# Autodesk Inventor assembly: Vex Traction Wheel 4x1
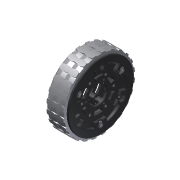
[picture p0: Inventor's stored thumbnail of the model, 180x180]
Saved by Autodesk Inventor 2013 (Build 170138000, 138)
## iProperties
Created: 2012-12-09
Part Number: Vex Traction Wheel 4x1
Document SubType Name: Assembly
Designer: Nemo
Mass: 137.424 g
Surface Area: 574.254 cm^2
Volume: 103.699 cm^3
Density: 1.32523 g/cm^3
Author: Nemo
## Documents named in this file (6)
- H:\Nemo\Documents\Robotics\COTS Parts\Wheels\VexPro Traction Wheels\Vex Traction Wheel 4x1.iam
- H:\Nemo\Documents\Robotics\COTS Parts\Wheels\VexPro Traction Wheels\Components\Traction Wheel Body 4in.ipt
- H:\Nemo\Documents\Robotics\COTS Parts\Fasteners\Hex Standoff 8-32 x750.ipt
- H:\Nemo\Documents\Robotics\COTS Parts\Fasteners\8-32 BHCS x1250.ipt
- H:\Nemo\Documents\Robotics\COTS Parts\Fasteners\8-32 locknut.ipt
- H:\Nemo\Documents\Robotics\COTS Parts\Wheels\VexPro Traction Wheels\Components\4 in Traction Tire.iam
## Components (16 placed, 5 different names)
1. Traction Wheel Body 4in:2 — Flush:1, Mate:2, Mate:4, Mate:5, Mate:6, Angle:1, Mate:7, Mate:8, Mate:9, Insert:4, Angle:3, Mate:11
2. Traction Wheel Body 4in:3 — Mate:5, Mate:8, Mate:9, Insert:3
3. 4 in Traction Tire:1 [sub-assembly] — Mate:10, Mate:11, Angle:4, Mate:13, Flush:2
4. 4 in Traction Tire:2 [sub-assembly] — Mate:12, Mate:13, Flush:2
5. Hex Standoff 8-32 x750:2 — Mate:6, Angle:1, Mate:7
6. Hex Standoff 8-32 x750:3
7. Hex Standoff 8-32 x750:4
8. Hex Standoff 8-32 x750:5
9. Hex Standoff 8-32 x750:6
10. Hex Standoff 8-32 x750:7
11. 8-32 BHCS x1250:1 — Insert:3
12. 8-32 locknut:2 — Insert:4, Angle:3
13. 8-32 BHCS x1250:3
14. 8-32 locknut:3
15. 8-32 BHCS x1250:5
16. 8-32 locknut:5
## Component patterns: (6 elements, first: Hex Standoff 8-32 x750:2), (3 elements, first: 8-32 BHCS x1250:1 + 8-32 locknut:2)
## Relationships (18: Mate 11, Angle 3, Flush 2, Insert 2)
- Flush:1: Traction Wheel Body 4in:2
- Mate:2: Traction Wheel Body 4in:2
- Mate:4: Traction Wheel Body 4in:2
- Mate:5: Traction Wheel Body 4in:2 ↔ Traction Wheel Body 4in:3
- Mate:6: Traction Wheel Body 4in:2 ↔ Hex Standoff 8-32 x750:2
- Angle:1 (0 deg): Traction Wheel Body 4in:2 ↔ Hex Standoff 8-32 x750:2
- Mate:7: Traction Wheel Body 4in:2 ↔ Hex Standoff 8-32 x750:2
- Mate:8: Traction Wheel Body 4in:2 ↔ Traction Wheel Body 4in:3
- Mate:9: Traction Wheel Body 4in:2 ↔ Traction Wheel Body 4in:3
- Insert:3: Traction Wheel Body 4in:3 ↔ 8-32 BHCS x1250:1
- Insert:4: Traction Wheel Body 4in:2 ↔ 8-32 locknut:2
- Angle:3 (0 deg): Traction Wheel Body 4in:2 ↔ 8-32 locknut:2
- Mate:10: 4 in Traction Tire:1
- Mate:11: Traction Wheel Body 4in:2 ↔ 4 in Traction Tire:1
- Angle:4 (15 deg): 4 in Traction Tire:1
- Mate:12: 4 in Traction Tire:2
- Mate:13: 4 in Traction Tire:1 ↔ 4 in Traction Tire:2
- Flush:2: 4 in Traction Tire:1 ↔ 4 in Traction Tire:2
